# Autodesk Inventor assembly: Tafel
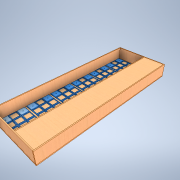
[picture p0: Inventor's stored thumbnail of the model, 180x180]
Saved by Autodesk Inventor 2021 (Build 250183000, 183)
## iProperties
Created: 2021-03-18
Part Number: Tafel
Document SubType Name: Assembly
Designer: ZiweZhang
Author: ZiweZhang
## Documents named in this file (8)
- E:\School\Projecten\Project 78 - Senstable\Design\Inventor\SensorTafel\Tafel.iam
- E:\School\Projecten\Project 78 - Senstable\Design\Inventor\SensorTafel\Binnenkant.ipt
- E:\School\Projecten\Project 78 - Senstable\Design\Inventor\SensorTafel\Bovenkant.ipt
- E:\School\Projecten\Project 78 - Senstable\Design\Inventor\SensorTafel\Linker-Rechterkanten.ipt
- E:\School\Projecten\Project 78 - Senstable\Design\Inventor\SensorTafel\Onderkant.ipt
- Onderkant.ipt
- E:\School\Projecten\Project 78 - Senstable\Design\Inventor\SensorTafel\Voor-Achterkant.ipt
- E:\School\Projecten\Project 78 - Senstable\Design\Inventor\SensorDoosje\Grid.ipt
## Components (13 placed, 6 different names)
1. Binnenkant:1 — Rigid:7
2. Bovenkant:1 — Rigid:6, Rigid:7
3. Linker-Rechterkanten:1 — Rigid:3, Rigid:6
4. Onderkant:1 — Rigid:1, Rigid:4, Rigid:8, Rigid:9, Rigid:10, Rigid:11, Rigid:12, Rigid:13
5. Voor-Achterkant:1 — Rigid:1, Rigid:3
6. Linker-Rechterkanten:2 — Rigid:5
7. Voor-Achterkant:2 — Rigid:4, Rigid:5
8. Grid:1 — Rigid:9
9. Grid:2 — Rigid:10
10. Grid:3 — Rigid:11
11. Grid:4 — Rigid:13
12. Grid:5 — Rigid:12
13. Grid:6 — Rigid:8
## Relationships (12: WeldJoint 12)
- Rigid:1 [WeldJoint]: Onderkant:1 ↔ Voor-Achterkant:1
- Rigid:3 [WeldJoint]: Linker-Rechterkanten:1 ↔ Voor-Achterkant:1
- Rigid:4 [WeldJoint]: Onderkant:1 ↔ Voor-Achterkant:2
- Rigid:5 [WeldJoint]: Linker-Rechterkanten:2 ↔ Voor-Achterkant:2
- Rigid:6 [WeldJoint]: Bovenkant:1 ↔ Linker-Rechterkanten:1
- Rigid:7 [WeldJoint]: Binnenkant:1 ↔ Bovenkant:1
- Rigid:8 [WeldJoint]: Onderkant:1 ↔ Grid:6
- Rigid:9 [WeldJoint]: Onderkant:1 ↔ Grid:1
- Rigid:10 [WeldJoint]: Onderkant:1 ↔ Grid:2
- Rigid:11 [WeldJoint]: Onderkant:1 ↔ Grid:3
- Rigid:12 [WeldJoint]: Onderkant:1 ↔ Grid:5
- Rigid:13 [WeldJoint]: Onderkant:1 ↔ Grid:4
